# Autodesk Inventor assembly: bracket_assy
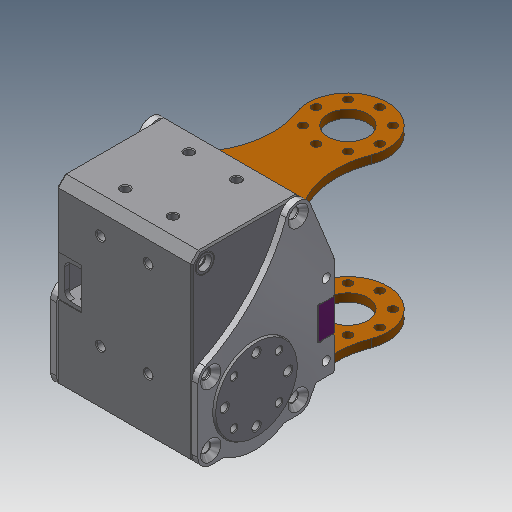
[picture p0: Inventor's stored thumbnail of the model, 512x512]
Saved by Autodesk Inventor 2019.4 (Build 234330000, 330)
## iProperties
Created: 2018-04-26
Part Number: bracket_assy
Material: 一般
Document SubType Name: Assembly
Designer: cmflab
Mass: 49.8802 g
Surface Area: 220.036 cm^2
Volume: 49.8802 cm^3
Density: 1 g/cm^3
Author: cmflab
## Documents named in this file (6)
- C:\Workspace\Yunit8-HaptHexa\Hardware\Inventor\Coxa\_Coxa.iam
- C:\Workspace\Yunit8-HaptHexa\Hardware\Inventor\Coxa\tap_block.ipt
- C:\Workspace\Yunit8-HaptHexa\Hardware\Inventor\Coxa\tab_yaw_top.ipt
- C:\Workspace\Yunit8-HaptHexa\Hardware\Inventor\Coxa\tab_pitch_out.ipt
- C:\Workspace\Yunit8-HaptHexa\Hardware\Inventor\X430\XL-430.iam
- C:\Workspace\Yunit8-HaptHexa\Hardware\Inventor\Coxa\tab_pitch_out_mir.ipt
## Components (6 placed, 5 different names)
1. tap_block:1 — メイト:1, メイト:2, メイト:3, メイト:4, メイト:5, メイト:6, メイト:7, メイト:8, メイト:9
2. tab_yaw_top:1 — メイト:1, メイト:2, メイト:6
3. tab_yaw_top:2 — メイト:4, メイト:5, メイト:3
4. tab_pitch_out:1 — メイト:7, メイト:8, メイト:9, メイト:10, メイト:11, メイト:12
5. tab_pitch_out_mir:1
6. XL-430:1 [sub-assembly] — メイト:10, メイト:11, メイト:12
## Relationships (12: Mate 12)
- メイト:1 [Mate]: tap_block:1 ↔ tab_yaw_top:1
- メイト:2 [Mate]: tap_block:1 ↔ tab_yaw_top:1
- メイト:3 [Mate]: tap_block:1 ↔ tab_yaw_top:2
- メイト:4 [Mate]: tap_block:1 ↔ tab_yaw_top:2
- メイト:5 [Mate]: tap_block:1 ↔ tab_yaw_top:2
- メイト:6 [Mate]: tap_block:1 ↔ tab_yaw_top:1
- メイト:7 [Mate]: tap_block:1 ↔ tab_pitch_out:1
- メイト:8 [Mate]: tap_block:1 ↔ tab_pitch_out:1
- メイト:9 [Mate]: tap_block:1 ↔ tab_pitch_out:1
- メイト:10 [Mate]: tab_pitch_out:1 ↔ XL-430:1
- メイト:11 [Mate]: tab_pitch_out:1 ↔ XL-430:1
- メイト:12 [Mate]: tab_pitch_out:1 ↔ XL-430:1
## Named parameters: sa_0 = 50, sa_1 = 2e-13, sa_2 = 500, sa_3 = 0
note: some values were not read from the file. Shown as the stored number, unit unknown: "sa_0", "sa_1", "sa_2", "sa_3".
